# Autodesk Inventor assembly: gyroGearHeadAssembly03
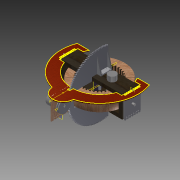
[picture p0: Inventor's stored thumbnail of the model, 180x180]
Saved by Autodesk Inventor 2013 (Build 170138000, 138)
## iProperties
Created: 2013-02-24
Part Number: gyroGearHeadAssembly03
Document SubType Name: Assembly
Designer: Nano
Author: Nano
## Documents named in this file (22)
- C:\Users\Nano\Documents\InventorByron\InventorMasterProject\gyroPhone01\gyroGearHeadAssembly03.iam
- C:\Users\Nano\Documents\InventorByron\InventorMasterProject\gyroPhone01\stepperMotorAndMount.iam
- C:\Users\Nano\Documents\InventorByron\InventorMasterProject\gyroPhone01\littleGear01.ipt
- C:\Users\Nano\Documents\InventorByron\InventorMasterProject\gyroPhone01\gearGuideRings.ipt
- C:\Users\Nano\Documents\InventorByron\InventorMasterProject\gyroPhone01\bigGearSection01.ipt
- C:\Users\Nano\Documents\InventorByron\InventorMasterProject\gyroPhone01\brace01.ipt
- C:\Users\Nano\Documents\InventorByron\InventorMasterProject\gyroPhone01\brace01_MIR1.ipt
- C:\Users\Nano\Documents\InventorByron\InventorMasterProject\gyroPhone01\brace02_MIR.ipt
- C:\Users\Nano\Documents\InventorByron\InventorMasterProject\gyroPhone01\basePlate01.ipt
- C:\Users\Nano\Documents\InventorByron\InventorMasterProject\gyroPhone01\basePlate01_MIR2.ipt
- C:\Users\Nano\Documents\InventorByron\InventorMasterProject\gyroPhone01\basePlate01_MIR3.ipt
- C:\Users\Nano\Documents\InventorByron\InventorMasterProject\gyroPhone01\basePlate01_MIR2_MIR.ipt
- C:\Users\Nano\Documents\InventorByron\InventorMasterProject\gyroPhone01\gyroWheelCradle01.ipt
- C:\Users\Nano\Documents\InventorByron\InventorMasterProject\gyroPhone01\shortEndAxel.ipt
- C:\Users\Nano\Documents\InventorByron\InventorMasterProject\gyroPhone01\shortEndAxel_MIR.ipt
- C:\Users\Nano\Documents\InventorByron\InventorMasterProject\gyroPhone01\wheelAxel01.ipt
- C:\Users\Nano\Documents\InventorByron\InventorMasterProject\gyroPhone01\motorWheelAssembly01.iam
- C:\Users\Nano\Documents\InventorByron\InventorMasterProject\gyroPhone01\gyroYoke01.ipt
- C:\Users\Nano\Documents\InventorByron\InventorMasterProject\gyroPhone01\yokeEndBlock.ipt
- C:\Users\Nano\Documents\InventorByron\InventorMasterProject\gyroPhone01\yokeEndBlock_MIR.ipt
- C:\Users\Nano\Documents\InventorByron\InventorMasterProject\gyroPhone01\stepperShaftCollar.ipt
- C:\Users\Nano\Documents\InventorByron\InventorMasterProject\gyroPhone01\gearAssemblyTake02\stepperMotorMountPlate01.ipt
## Components (22 placed, 21 different names)
1. stepperMotorAndMount:1 [sub-assembly] — Mate:1, Flush:1, Mate:2, Mate:4, Mate:8, Mate:9, Mate:28, Mate:29, Mate:31, Mate:32, Mate:33
2. Spur Gear1:1 — Mate:2, Mate:3, Mate:5, Mate:6, Mate:7, gearsFlushWithEachOther
3. gearGuideRings:1 — Mate:1, Flush:1, Mate:3, Mate:6
4. gearGuideRings:2 — Mate:4, Mate:5, Mate:7, Mate:30
5. Spur Gear2:1 — gearsFlushWithEachOther, Mate:8, Mate:9, Angle:1, Flush:3, Mate:10, Mate:11, Mate:12, Mate:13, Mate:14, Flush:4, Mate:16, Mate:17, Mate:18, Mate:19
6. brace01:1 — Flush:3, Mate:10, Mate:11, Mate:15
7. brace01_MIR1:1
8. brace02_MIR:1 — Mate:12, Mate:13, Mate:16
9. basePlate01:1 — Mate:14, Flush:4, Mate:15
10. basePlate01_MIR2:1
11. basePlate01_MIR3:1
12. basePlate01_MIR2_MIR:1
13. gyroWheelCradle01:1 — Mate:17, Mate:18, Mate:19, Mate:20, Flush:5, Mate:21, Flush:6, Mate:23, Flush:7, Mate:24, Mate:25
14. shortEndAxel:1 — Mate:20, Flush:5, Angle:2
15. shortEndAxel_MIR:1
16. wheelAxel01:1 — Mate:21, Flush:6, Mate:22
17. motorWheelAssembly01:1 [sub-assembly] — Mate:22, Mate:23, Angle:2
18. gyroYoke01:1 — Flush:7, Mate:24, Mate:25, Flush:8, Mate:26, Mate:27
19. yokeEndBlock:1 — Flush:8, Mate:26, Mate:27
20. yokeEndBlock_MIR:1
21. stepperShaftCollar:1 — Mate:28, Mate:29, Mate:30
22. stepperMotorMountPlate01:1 — Mate:31, Angle:1, Mate:32, Mate:33
## Relationships (43: Mate 33, Flush 8, Angle 2)
- Mate:1: stepperMotorAndMount:1 ↔ gearGuideRings:1
- Flush:1: stepperMotorAndMount:1 ↔ gearGuideRings:1
- Mate:2: stepperMotorAndMount:1 ↔ Spur Gear1:1
- Mate:3: Spur Gear1:1 ↔ gearGuideRings:1
- Mate:4: stepperMotorAndMount:1 ↔ gearGuideRings:2
- Mate:5: Spur Gear1:1 ↔ gearGuideRings:2
- Mate:6: Spur Gear1:1 ↔ gearGuideRings:1
- Mate:7: Spur Gear1:1 ↔ gearGuideRings:2
- gearsFlushWithEachOther [Flush]: Spur Gear1:1 ↔ Spur Gear2:1
- Mate:8 (196.1134 mm): stepperMotorAndMount:1 ↔ Spur Gear2:1
- Mate:9: stepperMotorAndMount:1 ↔ Spur Gear2:1
- Angle:1 (0 deg): Spur Gear2:1 ↔ stepperMotorMountPlate01:1
- Flush:3: Spur Gear2:1 ↔ brace01:1
- Mate:10: Spur Gear2:1 ↔ brace01:1
- Mate:11: Spur Gear2:1 ↔ brace01:1
- Mate:12: Spur Gear2:1 ↔ brace02_MIR:1
- Mate:13: Spur Gear2:1 ↔ brace02_MIR:1
- Mate:14: Spur Gear2:1 ↔ basePlate01:1
- Flush:4: Spur Gear2:1 ↔ basePlate01:1
- Mate:15: brace01:1 ↔ basePlate01:1
- Mate:16: Spur Gear2:1 ↔ brace02_MIR:1
- Mate:17: Spur Gear2:1 ↔ gyroWheelCradle01:1
- Mate:18: Spur Gear2:1 ↔ gyroWheelCradle01:1
- Mate:19: Spur Gear2:1 ↔ gyroWheelCradle01:1
- Mate:20: gyroWheelCradle01:1 ↔ shortEndAxel:1
- Flush:5: gyroWheelCradle01:1 ↔ shortEndAxel:1
- Mate:21: gyroWheelCradle01:1 ↔ wheelAxel01:1
- Flush:6: gyroWheelCradle01:1 ↔ wheelAxel01:1
- Mate:22: wheelAxel01:1 ↔ motorWheelAssembly01:1
- Mate:23 (5.5626 mm): gyroWheelCradle01:1 ↔ motorWheelAssembly01:1
- Angle:2 (0 deg): shortEndAxel:1 ↔ motorWheelAssembly01:1
- Flush:7: gyroWheelCradle01:1 ↔ gyroYoke01:1
- Mate:24 (3.175 mm): gyroWheelCradle01:1 ↔ gyroYoke01:1
- Mate:25 (6.35 mm): gyroWheelCradle01:1 ↔ gyroYoke01:1
- Flush:8: gyroYoke01:1 ↔ yokeEndBlock:1
- Mate:26: gyroYoke01:1 ↔ yokeEndBlock:1
- Mate:27: gyroYoke01:1 ↔ yokeEndBlock:1
- Mate:28: stepperMotorAndMount:1 ↔ stepperShaftCollar:1
- Mate:29 (3.175 mm): stepperMotorAndMount:1 ↔ stepperShaftCollar:1
- Mate:30: gearGuideRings:2 ↔ stepperShaftCollar:1
- Mate:31: stepperMotorAndMount:1 ↔ stepperMotorMountPlate01:1
- Mate:32: stepperMotorAndMount:1 ↔ stepperMotorMountPlate01:1
- Mate:33: stepperMotorAndMount:1 ↔ stepperMotorMountPlate01:1
